# Autodesk Inventor assembly: filterWheelAssembly
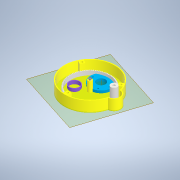
[picture p0: Inventor's stored thumbnail of the model, 180x180]
Saved by Autodesk Inventor 2022.1 (Build 261234020, 234B)
## iProperties
Created: 2020-04-12
Part Number: filterWheelAssembly
Document SubType Name: Assembly
Designer: robst
Author: robst
## Documents named in this file (10)
- C:\git\CAD-Development\robSteele\ShapeWays\TelescopeProjects\FilterWheel\filterWheelAssembly.iam
- C:\git\CAD-Development\robSteele\ShapeWays\TelescopeProjects\FilterWheel\filterBase.ipt
- C:\git\CAD-Development\robSteele\ShapeWays\TelescopeProjects\FilterWheel\filterHolder.ipt
- C:\git\CAD-Development\robSteele\ShapeWays\TelescopeProjects\FilterWheel\simulatedFilterWithoutThreads.ipt
- C:\git\CAD-Development\robSteele\ShapeWays\TelescopeProjects\FilterWheel\filterHolderBackPiece.ipt
- C:\git\CAD-Development\robSteele\ShapeWays\TelescopeProjects\FilterWheel\insertToScope.ipt
- C:\git\CAD-Development\robSteele\ShapeWays\TelescopeProjects\FilterWheel\filterTop.ipt
- c:\git\CAD-MfgResources\McMaster-Carr\BrassHeatSetInsertForPlastic\10-32 0_375 93365A156_HEAT-SET INSERTS FOR PLASTICS.ipt
- C:\git\CAD-Development\robSteele\ShapeWays\TelescopeProjects\FilterWheel\filterWheelAssembly\Design Accelerator\Spur Gears3.iam
- C:\Users\robst\Documents\Inventor\Content Center Files\R2021\en-US\U UNC 2605\Unbrako - 8 x 5_8 - 32(10).ipt
## Components (9 placed, 9 different names)
1. filterBase:1 — Insert:4, Insert:5, Insert:16, Insert:17
2. filterHolder:1 — Insert:1, Insert:3, Insert:4, Flush:1, Mate:23
3. simulatedFilterWithoutThreads:1 — Insert:1, Insert:2
4. filterHolderBackPiece:1 — Insert:2, Insert:3
5. insertToScope:1 — Insert:5
6. filterTop:1 — Insert:16, Mate:24, Mate:25
7. 10-32 0_375 93365A156_HEAT-SET INSERTS FOR PLASTICS:1 — Insert:17
8. Unbrako UNC Hex Socket Button Cap - Inch 8 x 5/8:1 — Mate:24, Mate:25
9. Spur Gears:1 [sub-assembly] — Mate:23, Flush:2
## Relationships (12: Insert 7, Mate 3, Flush 2)
- Insert:1: filterHolder:1 ↔ simulatedFilterWithoutThreads:1
- Insert:2: simulatedFilterWithoutThreads:1 ↔ filterHolderBackPiece:1
- Insert:3: filterHolder:1 ↔ filterHolderBackPiece:1
- Insert:4 (9.525 mm): filterBase:1 ↔ filterHolder:1
- Insert:5: filterBase:1 ↔ insertToScope:1
- Insert:16: filterBase:1 ↔ filterTop:1
- Insert:17: filterBase:1 ↔ 10-32 0_375 93365A156_HEAT-SET INSERTS FOR PLASTICS:1
- Flush:1: filterHolder:1
- Mate:23: filterHolder:1 ↔ Spur Gears:1
- Flush:2: Spur Gears:1
- Mate:24: filterTop:1 ↔ Unbrako UNC Hex Socket Button Cap - Inch 8 x 5/8:1
- Mate:25: filterTop:1 ↔ Unbrako UNC Hex Socket Button Cap - Inch 8 x 5/8:1
